# Autodesk Inventor assembly: 5mm Bearing Endcap
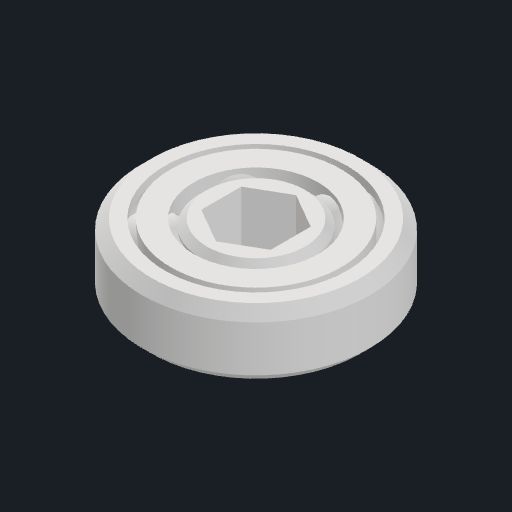
[picture p0: Inventor's stored thumbnail of the model, 512x512]
Saved by Autodesk Inventor 2023 (Build 270158000, 158)
## iProperties
Created: 2022-10-15
Part Number: 5mm Bearing Endcap
Document SubType Name: Assembly
Designer: izack
Author: izack
## Documents named in this file (5)
- G:\CAD Modeling\Private Robotics\Custom Tryhard Robot\Drivetrain\Swerve Module Parts\Bearing Parts\5mm Bearing Endcap.iam
- G:\CAD Modeling\Private Robotics\Custom Tryhard Robot\Drivetrain\Swerve Module Parts\Bearing Parts\4.5mm Ball Bearings.ipt
- G:\CAD Modeling\Private Robotics\Custom Tryhard Robot\Drivetrain\Swerve Module Parts\Bearing Parts\5mm Bearing Outside.ipt
- G:\CAD Modeling\Private Robotics\Custom Tryhard Robot\Drivetrain\Swerve Module Parts\Bearing Parts\Hex Bearing Spacer.ipt
- G:\CAD Modeling\Private Robotics\Custom Tryhard Robot\Drivetrain\Swerve Module Parts\Bearing Parts\5mm Hex Bearing Inside Blocker.ipt
## Components (8 placed, 4 different names)
1. 5mm Bearing Outside:1 — Flush:1, Mate:1, Flush:2, Flush:3, Mate:4
2. Hex Bearing Spacer:1 — Flush:1, Mate:1, Mate:3
3. 5mm Hex Bearing Inside Blocker:1 — Flush:2, Flush:3, Mate:4
4. 4.5mm Ball Bearings:1 — Mate:3
5. 4.5mm Ball Bearings:2
6. 4.5mm Ball Bearings:3
7. 4.5mm Ball Bearings:4
8. 4.5mm Ball Bearings:5
## Component patterns: (5 elements, first: 4.5mm Ball Bearings:1)
## Relationships (6: Flush 3, Mate 3)
- Flush:1: 5mm Bearing Outside:1 ↔ Hex Bearing Spacer:1
- Mate:1: 5mm Bearing Outside:1 ↔ Hex Bearing Spacer:1
- Mate:3: Hex Bearing Spacer:1 ↔ 4.5mm Ball Bearings:1
- Flush:2: 5mm Bearing Outside:1 ↔ 5mm Hex Bearing Inside Blocker:1
- Flush:3: 5mm Bearing Outside:1 ↔ 5mm Hex Bearing Inside Blocker:1
- Mate:4: 5mm Bearing Outside:1 ↔ 5mm Hex Bearing Inside Blocker:1
